# Autodesk Inventor assembly: s-assy-link1+2+3+4+5+gripper
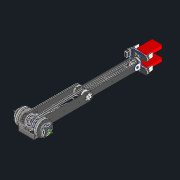
[picture p0: Inventor's stored thumbnail of the model, 180x180]
Saved by Autodesk Inventor 2021 (Build 250183000, 183)
## iProperties
Created: 2021-08-13
Part Number: s-assy-link1+2+3+4+5+gripper
Document SubType Name: Assembly
Designer: yuta0
Author: yuta0
## Documents named in this file (3)
- C:\Users\yuta0\Documents\GitHub\catchrobo_hardware\assy-robot\s-assy-link1+2+3+4+5+gripper.iam
- C:\Users\yuta0\Documents\GitHub\catchrobo_hardware\assy-robot\s-assy-link1.iam
- C:\Users\yuta0\Documents\GitHub\catchrobo_hardware\assy-robot\s-assy-link2+3+4+5+gripper.iam
## Components (2 placed, 2 different names)
1. s-assy-link1:1 [sub-assembly] — メイト:1, メイト:2
2. s-assy-link2+3+4+5+gripper:1 [sub-assembly] — メイト:1, メイト:2, 角度:1
## Relationships (3: Mate 2, Angle 1)
- メイト:1 [Mate]: s-assy-link1:1 ↔ s-assy-link2+3+4+5+gripper:1
- メイト:2 [Mate]: s-assy-link1:1 ↔ s-assy-link2+3+4+5+gripper:1
- 角度:1 [Angle] (270 deg): s-assy-link2+3+4+5+gripper:1
